# Autodesk Inventor assembly: 1444-17154_Aluminum_Chasis_Modification_MPSv2_V1
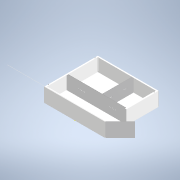
[picture p0: Inventor's stored thumbnail of the model, 180x180]
Saved by Autodesk Inventor 2021 (Build 250183000, 183)
## iProperties
Created: 2013-07-04
Part Number: 1444-17154_Aluminum_Chasis_Modification_MPSv2_V1
Document SubType Name: Assembly
Designer: Admin
Sending System: Autodesk Inventor 2013
Preprocessor: Autodesk Inventor 2013
Title: E:\Eng\Customer Service\Drawings\1444 & 1434\STEP Files\Conversion\1434-1715 & 1444-17154\1444-17154.iam.stp
## Documents named in this file (7)
- C:\Users\Barksdale\Dropbox (MIT)\MPI Group Folder\MPS\MPSV2\5xxx Enclosures\50xx Aluminum Chasis\5010_1444-17154_[DigiKey]_Aluminum_Chasis_Modification_MPSv2_V1.iam
- C:\Users\Barksdale\Dropbox (MIT)\MPI Group Folder\MPS\MPSV2\5xxx Enclosures\50xx Aluminum Chasis\500x Aluminum Chasis Parts [DigiKey]\1444-17154.ipt
- C:\Users\Barksdale\Dropbox (MIT)\MPI Group Folder\MPS\MPSV2\5xxx Enclosures\50xx Aluminum Chasis\500x Aluminum Chasis Parts [DigiKey]\1434-1715.ipt
- C:\Users\Barksdale\Dropbox (MIT)\MPI Group Folder\MPS\MPSV2\5xxx Enclosures\50xx Aluminum Chasis\500x Aluminum Chasis Parts [DigiKey]\6-32 (SC18394).ipt
- C:\Users\Barksdale\Dropbox (MIT)\MPI Group Folder\MPS\MPSV2\5xxx Enclosures\50xx Aluminum Chasis\5011_Aluminum_Chasis_Coil_Assembly_Tx_Filter_Separator_MPSv2_v1.ipt
- C:\Users\Barksdale\Dropbox (MIT)\MPI Group Folder\MPS\MPSV2\5xxx Enclosures\50xx Aluminum Chasis\5012_Aluminum_Chasis_Tx_Filter_Stage_Separator_MPSv2_v1.ipt
- C:\Users\Barksdale\Dropbox (MIT)\MPI Group Folder\MPS\MPSV2\5xxx Enclosures\50xx Aluminum Chasis\5013_Aluminum_Chasis_Coil_Assembly_Door_MPSv2_v1.ipt
## Components (8 placed, 6 different names)
1. 1444-17154:1 — Angle:1, Mate:1, Flush:1, Mate:2, Mate:3, Mate:4, Mate:6, Angle:2, Flush:2
2. 1434-1715:1 — Angle:1, Mate:1, Flush:1
3. 6-32 (SC18394):1
4. 6-32 (SC18394):2
5. 6-32 (SC18394):3
6. 5011_Aluminum_Chasis_Coil_Assembly_Tx_Filter_Separator_MPSv2_v1:1 — Mate:2, Mate:3, Mate:5
7. 5012_Aluminum_Chasis_Tx_Filter_Stage_Separator_MPSv2_v1:1 — Mate:4, Mate:5, Mate:6
8. 5013_Aluminum_Chasis_Coil_Assembly_Door_MPSv2_v1:1 — Angle:2, Flush:2
## Relationships (10: Mate 6, Angle 2, Flush 2)
- Angle:1 (135 deg): 1444-17154:1 ↔ 1434-1715:1
- Mate:1: 1444-17154:1 ↔ 1434-1715:1
- Flush:1: 1444-17154:1 ↔ 1434-1715:1
- Mate:2: 1444-17154:1 ↔ 5011_Aluminum_Chasis_Coil_Assembly_Tx_Filter_Separator_MPSv2_v1:1
- Mate:3: 1444-17154:1 ↔ 5011_Aluminum_Chasis_Coil_Assembly_Tx_Filter_Separator_MPSv2_v1:1
- Mate:4: 1444-17154:1 ↔ 5012_Aluminum_Chasis_Tx_Filter_Stage_Separator_MPSv2_v1:1
- Mate:5: 5011_Aluminum_Chasis_Coil_Assembly_Tx_Filter_Separator_MPSv2_v1:1 ↔ 5012_Aluminum_Chasis_Tx_Filter_Stage_Separator_MPSv2_v1:1
- Mate:6: 1444-17154:1 ↔ 5012_Aluminum_Chasis_Tx_Filter_Stage_Separator_MPSv2_v1:1
- Angle:2 (-45 deg): 1444-17154:1 ↔ 5013_Aluminum_Chasis_Coil_Assembly_Door_MPSv2_v1:1
- Flush:2: 1444-17154:1 ↔ 5013_Aluminum_Chasis_Coil_Assembly_Door_MPSv2_v1:1
